# Autodesk Inventor assembly: HS Bearing Flat with Screws
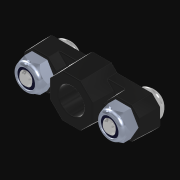
[picture p0: Inventor's stored thumbnail of the model, 180x180]
Saved by Autodesk Inventor 2021 (Build 250183000, 183)
## iProperties
Created: 2021-02-16
Part Number: HS Bearing Flat with Screws
Document SubType Name: Assembly
Designer: yuany
Author: yuany
## Documents named in this file (5)
- E:\VEX Cad\Library 1.2\Motion\HS Shaft\HS Bearing Flat with Screws.iam
- E:\VEX Cad\Library 1.2\Motion\HS Shaft\HS Bearing Flat.ipt
- E:\VEX Cad\Library 1.2\Structure\Hardware\Screw Steel - Hex\Screw 8-32 Steel .500.ipt
- E:\VEX Cad\Library 1.2\Structure\Hardware\Screw Steel - Hex.ipt
- E:\VEX Cad\Library 1.2\Structure\Hardware\Nut Thin Nylock.ipt
## Components (5 placed, 3 different names)
1. HS Bearing Flat:1 — Insert:1, Insert:2, Insert:3, Insert:4
2. Screw 8-32 Steel .500:1 — Insert:1
3. Screw 8-32 Steel .500:2 — Insert:2
4. Nut Thin Nylock:1 — Insert:4
5. Nut Thin Nylock:2 — Insert:3
## Relationships (4: Insert 4)
- Insert:1 (1.6002 mm): HS Bearing Flat:1 ↔ Screw 8-32 Steel .500:1
- Insert:2 (1.6002 mm): HS Bearing Flat:1 ↔ Screw 8-32 Steel .500:2
- Insert:3: HS Bearing Flat:1 ↔ Nut Thin Nylock:2
- Insert:4: HS Bearing Flat:1 ↔ Nut Thin Nylock:1
